# Autodesk Inventor assembly: CoreXY Idler 4040 Assembly Right
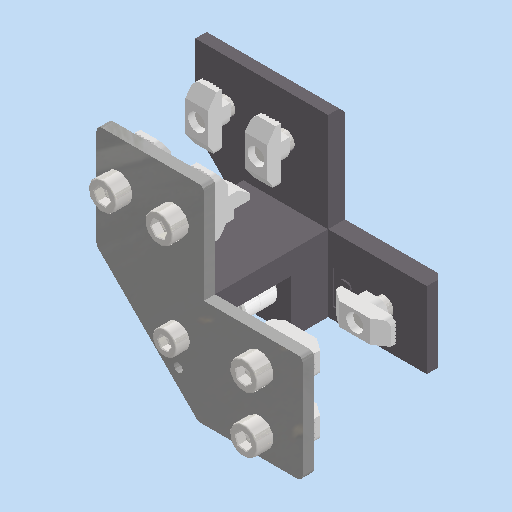
[picture p0: Inventor's stored thumbnail of the model, 512x512]
Saved by Autodesk Inventor 2023.2 (Build 272271000, 271)
## iProperties
Created: 2023-11-27
Part Number: CoreXY Idler 4040 Assembly Right
Document SubType Name: Assembly
Designer: Nils Bade
Author: Nils Bade
## Documents named in this file (13)
- C:\Users\nilsb\Documents\Inventor\Projektarbeit-Bade\RatRig_Bade\CoreXY Idler 4040 Assembly Right.iam
- C:\Users\nilsb\Documents\Inventor\Projektarbeit-Bade\RatRig_modified\xy Idler Right for 4040.ipt
- C:\Users\nilsb\Documents\Inventor\Projektarbeit-Bade\RatRig_modified\Idler Plate for 4040.ipt
- C:\Users\nilsb\Documents\Inventor\Projektarbeit-Bade\Schrauben\Cap Head Screw M5x55 v2.ipt
- C:\Users\nilsb\Documents\Inventor\Projektarbeit-Bade\RatRig_Standards\Hex Locking Nut - M5 v2.ipt
- C:\Users\nilsb\Documents\Inventor\Projektarbeit-Bade\RatRig_modified\T-NUT - DropIn 4040 SERIES - M6.ipt
- C:\Users\nilsb\Documents\Inventor\Projektarbeit-Bade\Schrauben\Cap Head Screw M6x16 - DIN912.ipt
- C:\Users\nilsb\Documents\Inventor\Projektarbeit-Bade\Schrauben\Cap Head Screw M6x12 v2.ipt
- C:\Users\nilsb\Documents\Inventor\Projektarbeit-Bade\Schrauben\Countersink Screw M6x14 v2.ipt
- C:\Users\nilsb\Documents\Inventor\Projektarbeit-Bade\RatRig_Standards\Mini Precision Shim - 8x5x1mm v2.ipt
- C:\Users\nilsb\Documents\Inventor\Projektarbeit-Bade\RatRig_Standards\Ball Bearing - F695ZZ v1.ipt
- C:\Users\nilsb\Documents\Inventor\Projektarbeit-Bade\RatRig_Standards\Ball Bearing - 695ZZ v1.ipt
- C:\Users\nilsb\Documents\Inventor\Projektarbeit-Bade\RatRig_Standards\Aluminium Spacer - 6mm v2.ipt
## Components (28 placed, 12 different names)
1. xy Idler Right for 4040:1 — Fluchtend:1, Fluchtend:2, Passend:1, Passend:5, Passend:9, Winkel:5, Passend:17, Passend:18, Winkel:7, Winkel:8, Winkel:9, Passend:22, Passend:23, Passend:24, Passend:26, Passend:27, Passend:36, Passend:38, Passend:39, Passend:41, Passend:42, Passend:43, Winkel:10
2. Idler Plate for 4040:1 — Fluchtend:1, Fluchtend:2, Passend:1, Passend:2, Passend:3, Passend:11, Passend:12, Passend:13, Passend:14, Winkel:1, Winkel:2, Winkel:3, Winkel:4, Passend:16, Passend:19, Passend:20, Passend:21, Passend:28, Passend:29, Passend:30, Passend:31, Passend:32, Passend:33, Passend:34, Passend:35, Passend:45
3. Cap Head Screw M5x55 v2:1 — Passend:2, Passend:3, Passend:4, Passend:44, Passend:46, Passend:48, Passend:50, Passend:52, Passend:55, Passend:56, Passend:57
4. Hex Locking Nut - M5 v2:1 — Passend:4, Passend:5, Winkel:10
5. T-NUT - DROP IN TYPE FOR 40 SERIES - M6:1 — Passend:11, Winkel:4, Passend:16
6. T-NUT - DROP IN TYPE FOR 40 SERIES - M6:2 — Passend:12, Winkel:3, Passend:19
7. T-NUT - DROP IN TYPE FOR 40 SERIES - M6:3 — Passend:13, Winkel:2, Passend:20
8. T-NUT - DROP IN TYPE FOR 40 SERIES - M6:4 — Passend:14, Winkel:1, Passend:21
9. T-NUT - DROP IN TYPE FOR 40 SERIES - M6:5 — Winkel:5, Passend:17, Passend:18
10. T-NUT - DROP IN TYPE FOR 40 SERIES - M6:6 — Passend:10, Winkel:9, Passend:22
11. T-NUT - DROP IN TYPE FOR 40 SERIES - M6:7 — Passend:9, Winkel:8, Passend:23
12. T-NUT - DROP IN TYPE FOR 40 SERIES - M6:9 — Passend:7, Winkel:7, Passend:24
13. Cap Head Screw M6x16 - DIN912:1 — Passend:26, Passend:27
14. Cap Head Screw M6x12 v2:1 — Passend:29, Passend:33
15. Cap Head Screw M6x12 v2:2 — Passend:28, Passend:32
16. Cap Head Screw M6x12 v2:3 — Passend:31, Passend:35
17. Cap Head Screw M6x12 v2:4 — Passend:30, Passend:34
18. Countersink Screw M6x14 v2:1 — Passend:38, Passend:42
19. Countersink Screw M6x14 v2:2 — Passend:39, Passend:43, Passend:10
20. Countersink Screw M6x14 v2:4 — Passend:36, Passend:41, Passend:7
21. Mini Precision Shim - 8x5x1mm v2:1 — Passend:44, Passend:45, Passend:54
22. Mini Precision Shim - 8x5x1mm v2:2 — Passend:52, Passend:53, Passend:58
23. Mini Precision Shim - 8x5x1mm v2:3 — Passend:57, Passend:60
24. Ball Bearing - F695ZZ v1:1 — Passend:50, Passend:51, Passend:53
25. Ball Bearing - F695ZZ v1:2 — Passend:46, Passend:49, Passend:54
26. Ball Bearing - 695ZZ v1:1 — Passend:48, Passend:49, Passend:51
27. Aluminium Spacer - 6mm v2:1 — Passend:56, Passend:59, Passend:60
28. Aluminium Spacer - 6mm v2:2 — Passend:55, Passend:58, Passend:59
## Relationships (64: Mate 53, Angle 9, Flush 2)
- Fluchtend:1 [Flush]: xy Idler Right for 4040:1 ↔ Idler Plate for 4040:1
- Fluchtend:2 [Flush]: xy Idler Right for 4040:1 ↔ Idler Plate for 4040:1
- Passend:1 [Mate]: xy Idler Right for 4040:1 ↔ Idler Plate for 4040:1
- Passend:2 [Mate]: Idler Plate for 4040:1 ↔ Cap Head Screw M5x55 v2:1
- Passend:3 [Mate]: Idler Plate for 4040:1 ↔ Cap Head Screw M5x55 v2:1
- Passend:4 [Mate]: Cap Head Screw M5x55 v2:1 ↔ Hex Locking Nut - M5 v2:1
- Passend:5 [Mate]: xy Idler Right for 4040:1 ↔ Hex Locking Nut - M5 v2:1
- Passend:7 [Mate]: T-NUT - DROP IN TYPE FOR 40 SERIES - M6:9 ↔ Countersink Screw M6x14 v2:4
- Passend:9 [Mate]: xy Idler Right for 4040:1 ↔ T-NUT - DROP IN TYPE FOR 40 SERIES - M6:7
- Passend:10 [Mate]: T-NUT - DROP IN TYPE FOR 40 SERIES - M6:6 ↔ Countersink Screw M6x14 v2:2
- Passend:11 [Mate]: Idler Plate for 4040:1 ↔ T-NUT - DROP IN TYPE FOR 40 SERIES - M6:1
- Passend:12 [Mate]: Idler Plate for 4040:1 ↔ T-NUT - DROP IN TYPE FOR 40 SERIES - M6:2
- Passend:13 [Mate]: Idler Plate for 4040:1 ↔ T-NUT - DROP IN TYPE FOR 40 SERIES - M6:3
- Passend:14 [Mate]: Idler Plate for 4040:1 ↔ T-NUT - DROP IN TYPE FOR 40 SERIES - M6:4
- Winkel:1 [Angle] (0 deg): Idler Plate for 4040:1 ↔ T-NUT - DROP IN TYPE FOR 40 SERIES - M6:4
- Winkel:2 [Angle] (0 deg): Idler Plate for 4040:1 ↔ T-NUT - DROP IN TYPE FOR 40 SERIES - M6:3
- Winkel:3 [Angle] (0 deg): Idler Plate for 4040:1 ↔ T-NUT - DROP IN TYPE FOR 40 SERIES - M6:2
- Winkel:4 [Angle] (0 deg): Idler Plate for 4040:1 ↔ T-NUT - DROP IN TYPE FOR 40 SERIES - M6:1
- Winkel:5 [Angle] (0 deg): xy Idler Right for 4040:1 ↔ T-NUT - DROP IN TYPE FOR 40 SERIES - M6:5
- Passend:16 [Mate] (5.5 mm): Idler Plate for 4040:1 ↔ T-NUT - DROP IN TYPE FOR 40 SERIES - M6:1
- Passend:17 [Mate]: xy Idler Right for 4040:1 ↔ T-NUT - DROP IN TYPE FOR 40 SERIES - M6:5
- Passend:18 [Mate] (5.5 mm): xy Idler Right for 4040:1 ↔ T-NUT - DROP IN TYPE FOR 40 SERIES - M6:5
- Passend:19 [Mate] (5.5 mm): Idler Plate for 4040:1 ↔ T-NUT - DROP IN TYPE FOR 40 SERIES - M6:2
- Passend:20 [Mate] (5.5 mm): Idler Plate for 4040:1 ↔ T-NUT - DROP IN TYPE FOR 40 SERIES - M6:3
- Passend:21 [Mate] (5.5 mm): Idler Plate for 4040:1 ↔ T-NUT - DROP IN TYPE FOR 40 SERIES - M6:4
- Winkel:7 [Angle] (0 deg): xy Idler Right for 4040:1 ↔ T-NUT - DROP IN TYPE FOR 40 SERIES - M6:9
- Winkel:8 [Angle] (0 deg): xy Idler Right for 4040:1 ↔ T-NUT - DROP IN TYPE FOR 40 SERIES - M6:7
- Winkel:9 [Angle] (0 deg): xy Idler Right for 4040:1 ↔ T-NUT - DROP IN TYPE FOR 40 SERIES - M6:6
- Passend:22 [Mate] (5.5 mm): xy Idler Right for 4040:1 ↔ T-NUT - DROP IN TYPE FOR 40 SERIES - M6:6
- Passend:23 [Mate] (5.5 mm): xy Idler Right for 4040:1 ↔ T-NUT - DROP IN TYPE FOR 40 SERIES - M6:7
- Passend:24 [Mate] (5.5 mm): xy Idler Right for 4040:1 ↔ T-NUT - DROP IN TYPE FOR 40 SERIES - M6:9
- Passend:26 [Mate]: xy Idler Right for 4040:1 ↔ Cap Head Screw M6x16 - DIN912:1
- Passend:27 [Mate]: xy Idler Right for 4040:1 ↔ Cap Head Screw M6x16 - DIN912:1
- Passend:28 [Mate]: Idler Plate for 4040:1 ↔ Cap Head Screw M6x12 v2:2
- Passend:29 [Mate]: Idler Plate for 4040:1 ↔ Cap Head Screw M6x12 v2:1
- Passend:30 [Mate]: Idler Plate for 4040:1 ↔ Cap Head Screw M6x12 v2:4
- Passend:31 [Mate]: Idler Plate for 4040:1 ↔ Cap Head Screw M6x12 v2:3
- Passend:32 [Mate]: Idler Plate for 4040:1 ↔ Cap Head Screw M6x12 v2:2
- Passend:33 [Mate]: Idler Plate for 4040:1 ↔ Cap Head Screw M6x12 v2:1
- Passend:34 [Mate]: Idler Plate for 4040:1 ↔ Cap Head Screw M6x12 v2:4
- Passend:35 [Mate]: Idler Plate for 4040:1 ↔ Cap Head Screw M6x12 v2:3
- Passend:36 [Mate]: xy Idler Right for 4040:1 ↔ Countersink Screw M6x14 v2:4
- Passend:38 [Mate]: xy Idler Right for 4040:1 ↔ Countersink Screw M6x14 v2:1
- Passend:39 [Mate]: xy Idler Right for 4040:1 ↔ Countersink Screw M6x14 v2:2
- Passend:41 [Mate]: xy Idler Right for 4040:1 ↔ Countersink Screw M6x14 v2:4
- Passend:42 [Mate]: xy Idler Right for 4040:1 ↔ Countersink Screw M6x14 v2:1
- Passend:43 [Mate]: xy Idler Right for 4040:1 ↔ Countersink Screw M6x14 v2:2
- Passend:44 [Mate]: Cap Head Screw M5x55 v2:1 ↔ Mini Precision Shim - 8x5x1mm v2:1
- Passend:45 [Mate]: Idler Plate for 4040:1 ↔ Mini Precision Shim - 8x5x1mm v2:1
- Passend:46 [Mate]: Cap Head Screw M5x55 v2:1 ↔ Ball Bearing - F695ZZ v1:2
- Passend:48 [Mate]: Cap Head Screw M5x55 v2:1 ↔ Ball Bearing - 695ZZ v1:1
- Passend:49 [Mate]: Ball Bearing - F695ZZ v1:2 ↔ Ball Bearing - 695ZZ v1:1
- Passend:50 [Mate]: Cap Head Screw M5x55 v2:1 ↔ Ball Bearing - F695ZZ v1:1
- Passend:51 [Mate]: Ball Bearing - F695ZZ v1:1 ↔ Ball Bearing - 695ZZ v1:1
- Passend:52 [Mate]: Cap Head Screw M5x55 v2:1 ↔ Mini Precision Shim - 8x5x1mm v2:2
- Passend:53 [Mate]: Mini Precision Shim - 8x5x1mm v2:2 ↔ Ball Bearing - F695ZZ v1:1
- Passend:54 [Mate]: Mini Precision Shim - 8x5x1mm v2:1 ↔ Ball Bearing - F695ZZ v1:2
- Passend:55 [Mate]: Cap Head Screw M5x55 v2:1 ↔ Aluminium Spacer - 6mm v2:2
- Passend:56 [Mate]: Cap Head Screw M5x55 v2:1 ↔ Aluminium Spacer - 6mm v2:1
- Passend:57 [Mate]: Cap Head Screw M5x55 v2:1 ↔ Mini Precision Shim - 8x5x1mm v2:3
- Passend:58 [Mate]: Mini Precision Shim - 8x5x1mm v2:2 ↔ Aluminium Spacer - 6mm v2:2
- Passend:59 [Mate]: Aluminium Spacer - 6mm v2:1 ↔ Aluminium Spacer - 6mm v2:2
- Passend:60 [Mate]: Mini Precision Shim - 8x5x1mm v2:3 ↔ Aluminium Spacer - 6mm v2:1
- Winkel:10 [Angle] (0 deg): xy Idler Right for 4040:1 ↔ Hex Locking Nut - M5 v2:1
